# Autodesk Inventor assembly: MotorBoard_V1.0_Dribbler
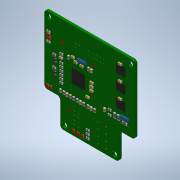
[picture p0: Inventor's stored thumbnail of the model, 180x180]
Saved by Autodesk Inventor 2020 (Build 240168000, 168)
## iProperties
Created: 2019-05-21
Part Number: MotorBoard_V1.0_Dribbler
Document SubType Name: Assembly
Designer: jg_ma
Sending System: Autodesk Translation Framework v8.2.0.1029
Preprocessor: ST-DEVELOPER v18
Title: c:\worker\convert-fusion-r04\tmp\job-1\22\output\files\b872785a-0138-4be1-bd62-03ee52a1c504\7be4d94e-0292-4e32-a0a1-3c0b01f39913.stp
## Documents named in this file (4)
- G:\Meu Drive\RobôCIn\Mecânica\SSL\2021\Inventor\first_floor\Components\MotorBoard\MOTORBOARD_V1.0_DRIBBLER.IAM
- G:\Meu Drive\RobôCIn\Mecânica\SSL\2021\Inventor\first_floor\Components\MotorBoard\PCB Component.iam
- G:\Meu Drive\RobôCIn\Mecânica\SSL\2021\Inventor\first_floor\Components\MotorBoard\559592030.ipt
- G:\Meu Drive\RobôCIn\Mecânica\SSL\2021\Inventor\first_floor\Components\MotorBoard\039281083.ipt
## Components (3 placed, 3 different names)
1. PCB Component:1 [sub-assembly] — Mate:1, Flush:1, Mate:2, Flush:2
2. 559592030:1 — Mate:1, Flush:1
3. 039281083:1 — Mate:2, Flush:2
## Relationships (4: Mate 2, Flush 2)
- Mate:1: PCB Component:1 ↔ 559592030:1
- Flush:1: PCB Component:1 ↔ 559592030:1
- Mate:2: PCB Component:1 ↔ 039281083:1
- Flush:2 (1 mm): PCB Component:1 ↔ 039281083:1
